# Autodesk Inventor assembly: ParisTruck
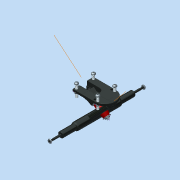
[picture p0: Inventor's stored thumbnail of the model, 180x180]
Saved by Autodesk Inventor 2015 (Build 190159000, 159)
## iProperties
Created: 2015-11-06
Part Number: ParisTruck
Document SubType Name: Assembly
Designer: Raphael
Author: Joey
Sending System: NX 8.0.0.25
Author: Raphael
## Documents named in this file (12)
- \\psf\Home\Documents\electric-skateboard\CAD\ParisTruck.iam
- \\psf\Home\Documents\electric-skateboard\CAD\Extra Hardware (Nut).ipt
- \\psf\Home\Documents\electric-skateboard\CAD\Nut.ipt
- \\psf\Home\Documents\electric-skateboard\CAD\Kingpin Nut.ipt
- \\psf\Home\Documents\electric-skateboard\CAD\Screw.ipt
- \\psf\Home\Documents\electric-skateboard\CAD\Roadside Washer.ipt
- \\psf\Home\Documents\electric-skateboard\CAD\Boardside Bushing.ipt
- \\psf\Home\Documents\electric-skateboard\CAD\Roadside Bushing.ipt
- \\psf\Home\Documents\electric-skateboard\CAD\Washer.ipt
- \\psf\Home\Documents\electric-skateboard\CAD\Paris Trucks.ipt
- \\psf\Home\Documents\electric-skateboard\CAD\Baseplate.ipt
- \\psf\Home\Documents\electric-skateboard\CAD\Baseplate Nut.ipt
## Components (17 placed, 11 different names)
1. Extra Hardware (Nut) — Mate:7, Mate:8
2. Extra Hardware (Nut):1 — Mate:3, Mate:4
3. Extra Hardware (Nut):2 — Mate:13, Mate:14
4. Extra Hardware (Nut):3 — Mate:15, Mate:16
5. Nut — Mate:25, Flush:1
6. Kingpin Nut — Mate:17, Mate:22
7. Screw — Mate:1, Mate:2, Mate:3
8. Screw:1 — Mate:9, Mate:10, Mate:13
9. Screw:2 — Mate:5, Mate:6, Mate:7
10. Roadside Washer — Mate:18, Mate:22, Mate:23
11. Boardside Bushing — Mate:19, Mate:30, Mate:31, Mate:32, Mate:33, Mate:41
12. Roadside Bushing — Mate:17, Mate:18, Mate:19, Mate:23, Mate:30
13. Washer — Mate:31, Mate:32, Mate:35
14. Screw:3 — Mate:11, Mate:12, Mate:15
15. Paris Trucks — Mate:25, Flush:1, Mate:40, Flush:2, Mate:41, Mate:43, Mate:46, Angle:2
16. Baseplate — Mate:1, Mate:2, Mate:4, Mate:5, Mate:6, Mate:8, Mate:9, Mate:10, Mate:11, Mate:12, Mate:14, Mate:16, Mate:33, Mate:35, Mate:37, Angle:2, Mate:47
17. Baseplate Nut — Mate:40, Flush:2
## Relationships (38: Mate 34, Flush 2, Angle 2)
- Mate:1: Screw ↔ Baseplate
- Mate:2 (12 mm): Screw ↔ Baseplate
- Mate:3: Extra Hardware (Nut):1 ↔ Screw
- Mate:4: Extra Hardware (Nut):1 ↔ Baseplate
- Mate:5: Screw:2 ↔ Baseplate
- Mate:6 (12 mm): Screw:2 ↔ Baseplate
- Mate:7: Extra Hardware (Nut) ↔ Screw:2
- Mate:8: Extra Hardware (Nut) ↔ Baseplate
- Mate:9: Screw:1 ↔ Baseplate
- Mate:10 (12 mm): Screw:1 ↔ Baseplate
- Mate:11 (12 mm): Screw:3 ↔ Baseplate
- Mate:12: Screw:3 ↔ Baseplate
- Mate:13: Extra Hardware (Nut):2 ↔ Screw:1
- Mate:14: Extra Hardware (Nut):2 ↔ Baseplate
- Mate:15: Extra Hardware (Nut):3 ↔ Screw:3
- Mate:16: Extra Hardware (Nut):3 ↔ Baseplate
- Mate:17: Kingpin Nut ↔ Roadside Bushing
- Mate:18: Roadside Washer ↔ Roadside Bushing
- Mate:19: Boardside Bushing ↔ Roadside Bushing
- Mate:22: Kingpin Nut ↔ Roadside Washer
- Mate:23: Roadside Washer ↔ Roadside Bushing
- Mate:25: Nut ↔ Paris Trucks
- Flush:1: Nut ↔ Paris Trucks
- Mate:30 (7.9375 mm): Boardside Bushing ↔ Roadside Bushing
- Mate:31: Boardside Bushing ↔ Washer
- Mate:32: Boardside Bushing ↔ Washer
- Mate:33: Boardside Bushing ↔ Baseplate
- Mate:35: Washer ↔ Baseplate
- Mate:37: Baseplate
- Mate:40: Paris Trucks ↔ Baseplate Nut
- Flush:2: Paris Trucks ↔ Baseplate Nut
- Mate:41: Boardside Bushing ↔ Paris Trucks
- Mate:43: Paris Trucks
- Mate:45
- Angle:1 (0 deg)
- Mate:46: Paris Trucks
- Angle:2 (90 deg): Paris Trucks ↔ Baseplate
- Mate:47: Baseplate
